# Autodesk Inventor assembly: engre certo
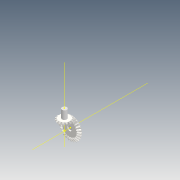
[picture p0: Inventor's stored thumbnail of the model, 180x180]
Saved by Autodesk Inventor 2021 (Build 250183000, 183)
## iProperties
Created: 2020-10-13
Part Number: engre certo
Document SubType Name: Assembly
Designer: evert
Author: evert
## Documents named in this file (4)
- C:\Users\evert\OneDrive\Área de Trabalho\peca move\engre certo.iam
- C:\Users\evert\OneDrive\Área de Trabalho\peca move\engre certo\Design Accelerator\Engrenagens cônicas2.iam
- C:\Users\evert\OneDrive\Área de Trabalho\peca move\Peçaasdasdadadda.ipt
- C:\Users\evert\OneDrive\Área de Trabalho\peca move\sup engrenagem menor.ipt
## Components (3 placed, 3 different names)
1. Engrenagens cônicas:1 [sub-assembly] — Rígida:1, Rotativa:1
2. Peçaasdasdadadda:1 — Rígida:1
3. sup engrenagem menor:1 — Rotativa:1
## Relationships (2: WeldJoint 1, RevoluteJoint 1)
- Rígida:1 [WeldJoint]: Engrenagens cônicas:1 ↔ Peçaasdasdadadda:1
- Rotativa:1 [RevoluteJoint]: Engrenagens cônicas:1 ↔ sup engrenagem menor:1
